# Autodesk Inventor assembly: Estante Pequeño
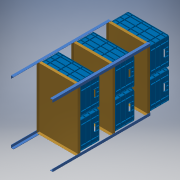
[picture p0: Inventor's stored thumbnail of the model, 180x180]
Saved by Autodesk Inventor 2016 (Build 200138000, 138)
## iProperties
Created: 2015-11-20
Part Number: Estante Pequeño
Material: Genérico
Document SubType Name: Assembly
Designer: David
_SolveAssemblyDoc: Frame Generator Solve Assembly
_Version: 15.0.0
Author: David
## Documents named in this file (5)
- D:\Programas\xampp\htdocs\localUnal\storage\macros\cuarto\Modelado\estantería\Estante Pequeño\Estante Pequeño.iam
- D:\Programas\xampp\htdocs\localUnal\storage\macros\cuarto\Modelado\estantería\Estante Pequeño\Esqueleto Pequeño.ipt
- D:\Programas\xampp\htdocs\localUnal\storage\macros\cuarto\Modelado\estantería\Estante Pequeño\Estante Pequeño\Frame\Frame0001.iam
- D:\Programas\xampp\htdocs\localUnal\storage\macros\cuarto\Modelado\estantería\estantería\lámina.ipt
- D:\Programas\xampp\htdocs\localUnal\storage\macros\cuarto\Modelado\estantería\Storage Bin 50L.ipt
## Components (11 placed, 4 different names)
1. Esqueleto Pequeño:1
2. Frame0001:1 [sub-assembly] — Coincidencia:1, Coincidencia:2, Nivelación:1, Coincidencia:3, Coincidencia:5, Coincidencia:6
3. lámina:1 — Coincidencia:1, Coincidencia:2, Nivelación:1, Coincidencia:4
4. lámina:2
5. lámina:3
6. Storage Bin 50L:2 — Nivelación:2, Nivelación:3, Coincidencia:6
7. Storage Bin 50L:1 — Coincidencia:3, Coincidencia:4, Coincidencia:5, Nivelación:2, Nivelación:3
8. Storage Bin 50L:3
9. Storage Bin 50L:4
10. Storage Bin 50L:5
11. Storage Bin 50L:6
## Component patterns: (3 elements, first: lámina:1), (3 elements, first: Storage Bin 50L:2 + Storage Bin 50L:1)
## Relationships (9: Mate 6, Flush 3)
- Coincidencia:1 [Mate]: Frame0001:1 ↔ lámina:1
- Coincidencia:2 [Mate]: Frame0001:1 ↔ lámina:1
- Nivelación:1 [Flush]: Frame0001:1 ↔ lámina:1
- Coincidencia:3 [Mate]: Frame0001:1 ↔ Storage Bin 50L:1
- Coincidencia:4 [Mate]: lámina:1 ↔ Storage Bin 50L:1
- Coincidencia:5 [Mate]: Frame0001:1 ↔ Storage Bin 50L:1
- Nivelación:2 [Flush]: Storage Bin 50L:2 ↔ Storage Bin 50L:1
- Nivelación:3 [Flush]: Storage Bin 50L:2 ↔ Storage Bin 50L:1
- Coincidencia:6 [Mate]: Frame0001:1 ↔ Storage Bin 50L:2
